# Autodesk Inventor assembly: inner_guide_asm
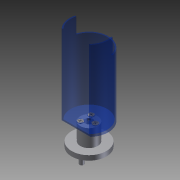
[picture p0: Inventor's stored thumbnail of the model, 180x180]
Saved by Autodesk Inventor 2011 SP2 (Build 150309200, 309)
## iProperties
Created: 2012-05-25
Part Number: inner_guide_asm
Document SubType Name: Assembly
Designer: sungwook
Author: sungwook
## Documents named in this file (4)
- C:\Users\sungwook\Documents\Inventor\Micron20_Base_Tube_Adjst\05222012_Inner_Guide_Tube\inner_guide_asm.iam
- C:\Users\sungwook\Documents\Inventor\Micron20_Base_Tube_Adjst\05222012_Inner_Guide_Tube\ss_inner_guide_top.ipt
- C:\Users\sungwook\Documents\Inventor\Micron20_Base_Tube_Adjst\05222012_Inner_Guide_Tube\ss_inner_guide_bottom.ipt
- C:\Users\sungwook\Documents\Inventor\Content Center Files\R2011\en-US\ANSI B18.6.3(00)\ANSI B18.6.3 - 2-56 UNC - 0.1875(32).ipt
## Components (5 placed, 3 different names)
1. ss_inner_guide_top:1 — Flush:1, Mate:2, Mate:3, Mate:4, Mate:6
2. ss_inner_guide_bottom:1 — Flush:1, Mate:2, Mate:3, Mate:4, Mate:5
3. Cross Recessed 100° Flat Countersunk Head Machine Screw - Type I - Inch 2-56 UNC x 0.1875:1 — Mate:5, Mate:6
4. Cross Recessed 100° Flat Countersunk Head Machine Screw - Type I - Inch 2-56 UNC x 0.1875:2
5. Cross Recessed 100° Flat Countersunk Head Machine Screw - Type I - Inch 2-56 UNC x 0.1875:3
## Component patterns: (3 elements, first: Cross Recessed 100° Flat Countersunk Head Machine Screw - Type I - Inch 2-56 UNC x 0.1875:1)
## Relationships (6: Mate 5, Flush 1)
- Flush:1: ss_inner_guide_top:1 ↔ ss_inner_guide_bottom:1
- Mate:2: ss_inner_guide_top:1 ↔ ss_inner_guide_bottom:1
- Mate:3: ss_inner_guide_top:1 ↔ ss_inner_guide_bottom:1
- Mate:4: ss_inner_guide_top:1 ↔ ss_inner_guide_bottom:1
- Mate:6: ss_inner_guide_top:1 ↔ Cross Recessed 100° Flat Countersunk Head Machine Screw - Type I - Inch 2-56 UNC x 0.1875:1
- Mate:5: ss_inner_guide_bottom:1 ↔ Cross Recessed 100° Flat Countersunk Head Machine Screw - Type I - Inch 2-56 UNC x 0.1875:1
